# Autodesk Inventor assembly: CH-2-01-Chassis Assembly
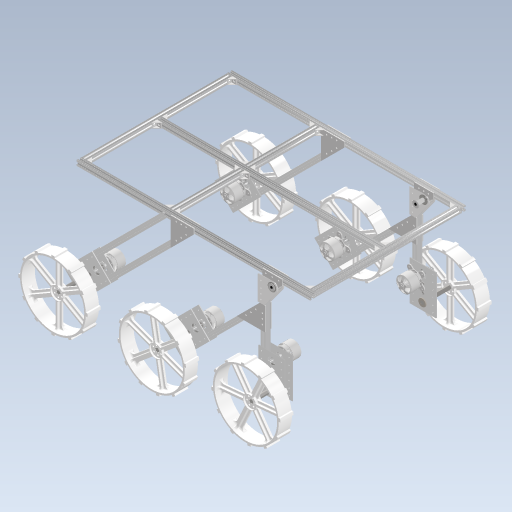
[picture p0: Inventor's stored thumbnail of the model, 512x512]
Saved by Autodesk Inventor 2023 (Build 270158000, 158)
## iProperties
Created: 2023-02-17
Part Number: CH-2-01-Chassis Assembly
Document SubType Name: Assembly
Designer: Dave
Author: Dave
## Documents named in this file (9)
- C:\Users\Dave\Documents\GitHub\BehrendURCMechanical\CAD\Chassis\CH-2-01-Chassis Assembly.iam
- C:\Users\Dave\Documents\GitHub\BehrendURCMechanical\CAD\Chassis\GearBox\Final Gears and Assemblies\FrontGearboxAssembly.iam
- C:\Users\Dave\Documents\GitHub\BehrendURCMechanical\CAD\Chassis\GearBox\Final Gears and Assemblies\RearGearboxAssembly.iam
- C:\Users\Dave\Documents\GitHub\BehrendURCMechanical\CAD\Chassis\CH-1-01-BearingBracket.ipt
- C:\Users\Dave\Documents\GitHub\BehrendURCMechanical\CAD\Chassis\GearBox\Final Gears and Assemblies\FrontGearboxAssembly_MIR.iam
- C:\Users\Dave\Documents\GitHub\BehrendURCMechanical\CAD\Chassis\GearBox\Final Gears and Assemblies\RearGearboxAssembly_MIR.iam
- C:\Users\Dave\Documents\GitHub\BehrendURCMechanical\CAD\Chassis\Ch-0-02-ChassisFrame.iam
- C:\Users\Dave\Documents\GitHub\BehrendURCMechanical\CAD\Chassis\6-Spoke Wheel.ipt
- C:\Users\Dave\Documents\GitHub\BehrendURCMechanical\CAD\Chassis\CH-1-02-BearingBracket.ipt
## Components (13 placed, 8 different names)
1. FrontGearboxAssembly:1 [sub-assembly] — Mate:5, Mate:15, Flush:16, Flush:17, Mate:21, Mate:22, Angle:2, Flush:20
2. RearGearboxAssembly:1 [sub-assembly] — Tangent:1, Flush:8, Mate:10, Flush:12, Flush:18, Mate:20
3. Ch-0-02-ChassisFrame:1 [sub-assembly] — Mate:9, Mate:10, Mate:12, Mate:13, Mate:14, Mate:15, Mate:16, Flush:11, Flush:12, Tangent:3, Tangent:4, Angle:2, Flush:19, Mate:23
4. CH-1-01-BearingBracket:1 — Mate:5, Mate:12, Mate:13
5. FrontGearboxAssembly_MIR:1 [sub-assembly] — Mate:14, Tangent:4, Flush:13, Flush:14, Mate:18, Mate:19, Mate:24, Flush:20
6. RearGearboxAssembly_MIR:1 [sub-assembly] — Tangent:2, Flush:8, Mate:9, Mate:16, Flush:11, Tangent:3, Flush:15, Mate:17
7. CH-1-02-BearingBracket:1 — Flush:19, Mate:23, Mate:24
8. 6-Spoke Wheel:1 — Flush:15, Mate:17
9. 6-Spoke Wheel:2 — Flush:14, Mate:18
10. 6-Spoke Wheel:3 — Flush:13, Mate:19
11. 6-Spoke Wheel:4 — Flush:16, Mate:22
12. 6-Spoke Wheel:5 — Flush:17, Mate:21
13. 6-Spoke Wheel:6 — Flush:18, Mate:20
## Relationships (35: Mate 16, Flush 14, Tangent 4, Angle 1)
- [Flush]: Ch-0-02-ChassisFrame:1
- [Flush]: Ch-0-02-ChassisFrame:1
- [Flush]: Ch-0-02-ChassisFrame:1
- Tangent:1: RearGearboxAssembly:1
- Mate:5: FrontGearboxAssembly:1 ↔ CH-1-01-BearingBracket:1
- Tangent:2: RearGearboxAssembly_MIR:1
- Flush:8: RearGearboxAssembly:1 ↔ RearGearboxAssembly_MIR:1
- Mate:9: Ch-0-02-ChassisFrame:1 ↔ RearGearboxAssembly_MIR:1
- Mate:10: RearGearboxAssembly:1 ↔ Ch-0-02-ChassisFrame:1
- Mate:12: Ch-0-02-ChassisFrame:1 ↔ CH-1-01-BearingBracket:1
- Mate:13: Ch-0-02-ChassisFrame:1 ↔ CH-1-01-BearingBracket:1
- Mate:14: Ch-0-02-ChassisFrame:1 ↔ FrontGearboxAssembly_MIR:1
- Mate:15: FrontGearboxAssembly:1 ↔ Ch-0-02-ChassisFrame:1
- Mate:16: Ch-0-02-ChassisFrame:1 ↔ RearGearboxAssembly_MIR:1
- Flush:11: Ch-0-02-ChassisFrame:1 ↔ RearGearboxAssembly_MIR:1
- Flush:12: RearGearboxAssembly:1 ↔ Ch-0-02-ChassisFrame:1
- Tangent:3: Ch-0-02-ChassisFrame:1 ↔ RearGearboxAssembly_MIR:1
- Tangent:4 (127 mm): Ch-0-02-ChassisFrame:1 ↔ FrontGearboxAssembly_MIR:1
- Flush:13: FrontGearboxAssembly_MIR:1 ↔ 6-Spoke Wheel:3
- Flush:14: FrontGearboxAssembly_MIR:1 ↔ 6-Spoke Wheel:2
- Flush:15: RearGearboxAssembly_MIR:1 ↔ 6-Spoke Wheel:1
- Mate:17: RearGearboxAssembly_MIR:1 ↔ 6-Spoke Wheel:1
- Mate:18: FrontGearboxAssembly_MIR:1 ↔ 6-Spoke Wheel:2
- Mate:19: FrontGearboxAssembly_MIR:1 ↔ 6-Spoke Wheel:3
- Flush:16: FrontGearboxAssembly:1 ↔ 6-Spoke Wheel:4
- Flush:17: FrontGearboxAssembly:1 ↔ 6-Spoke Wheel:5
- Flush:18: RearGearboxAssembly:1 ↔ 6-Spoke Wheel:6
- Mate:20: RearGearboxAssembly:1 ↔ 6-Spoke Wheel:6
- Mate:21: FrontGearboxAssembly:1 ↔ 6-Spoke Wheel:5
- Mate:22: FrontGearboxAssembly:1 ↔ 6-Spoke Wheel:4
- Angle:2 (0 deg): FrontGearboxAssembly:1 ↔ Ch-0-02-ChassisFrame:1
- Flush:19: Ch-0-02-ChassisFrame:1 ↔ CH-1-02-BearingBracket:1
- Mate:23: Ch-0-02-ChassisFrame:1 ↔ CH-1-02-BearingBracket:1
- Mate:24: FrontGearboxAssembly_MIR:1 ↔ CH-1-02-BearingBracket:1
- Flush:20: FrontGearboxAssembly:1 ↔ FrontGearboxAssembly_MIR:1
